# Autodesk Inventor assembly: satu
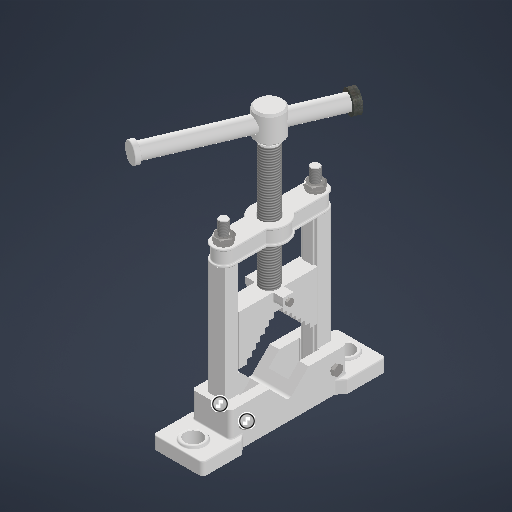
[picture p0: Inventor's stored thumbnail of the model, 512x512]
Saved by Autodesk Inventor 2026.1 (Build 301233000, 233)
## iProperties
Created: 2025-09-15
Part Number: satu
Document SubType Name: Assembly
Designer: student
Author: student
## Documents named in this file (13)
- C:\Users\student\Documents\satu\satu.iam
- C:\Users\student\Documents\satu\alaptest.ipt
- C:\Users\student\Documents\satu\menetesorso.ipt
- C:\Users\student\Documents\satu\oszlop.ipt
- C:\Users\student\Documents\satu\osszekotoelem.ipt
- C:\Users\student\Documents\satu\pfa.ipt
- C:\Users\student\Documents\satu\1.ipt
- C:\Users\student\Documents\Inventor\Content Center Files\R2026\en-US\BS 4464\BS 4464 - 10,6.ipt
- C:\Users\student\Documents\Inventor\Content Center Files\R2026\en-US\DIN 439-2\DIN 439 - M10 x 1,5.ipt
- C:\Users\student\Documents\Inventor\Content Center Files\R2026\en-US\AS 1110\AS 1110 - M6 x 50.ipt
- C:\Users\student\Documents\Inventor\Content Center Files\R2026\en-US\AS 1110\AS 1110 - M4 x 8.ipt
- C:\Users\student\Documents\Inventor\Content Center Files\R2026\en-US\ISO 4034(2)\ISO 4034 - M6 - ISO.ipt
- C:\Users\student\Documents\Inventor\Content Center Files\R2026\en-US\DIN 7989-2\DIN 7989 - 12_ - A.ipt
## Components (18 placed, 12 different names)
1. alaptest:1 — Mate:1, Mate:2, Mate:3, Mate:4, Mate:5, Mate:6, Insert:1, Insert:2, Mate:24, Mate:26
2. menetesorso:1 — Mate:10, Mate:11, Mate:12, Tangent:1, Mate:14
3. oszlop:1 — Mate:1, Mate:2, Mate:3, Mate:7, Mate:9, Mate:15, Mate:21
4. osszekotoelem:1 — Mate:7, Mate:8, Mate:9, Mate:10, Mate:14, Mate:16, Mate:18
5. pfa:1 — Mate:12, Mate:13, Tangent:1, Insert:3, Insert:4
6. 1:1 — Mate:11, Mate:27, Mate:28
7. oszlop:2 — Mate:4, Mate:5, Mate:6, Mate:8, Mate:13, Mate:17, Mate:19
8. BS 4464 10,6:1 — Mate:15, Mate:16, Mate:22
9. BS 4464 10,6:2 — Mate:17, Mate:18, Mate:20
10. DIN 439-2 - replaced by DIN EN 24035/28675 M10:1 — Mate:19, Mate:20
11. DIN 439-2 - replaced by DIN EN 24035/28675 M10:2 — Mate:21, Mate:22
12. AS 1110 - Metric M6 x 50:1 — Insert:1, Mate:25
13. AS 1110 - Metric M6 x 50:2 — Insert:2, Mate:23
14. AS 1110 - Metric M4 x 8:1 — Insert:3
15. AS 1110 - Metric M4 x 8:2 — Insert:4
16. ISO 4034 M6:1 — Mate:23, Mate:24
17. ISO 4034 M6:2 — Mate:25, Mate:26
18. DIN 7989-2 12" - A:1 — Mate:27, Mate:28
## Relationships (33: Mate 28, Insert 4, Tangent 1)
- Mate:1: alaptest:1 ↔ oszlop:1
- Mate:2: alaptest:1 ↔ oszlop:1
- Mate:3: alaptest:1 ↔ oszlop:1
- Mate:4: alaptest:1 ↔ oszlop:2
- Mate:5: alaptest:1 ↔ oszlop:2
- Mate:6: alaptest:1 ↔ oszlop:2
- Mate:7: oszlop:1 ↔ osszekotoelem:1
- Mate:8: osszekotoelem:1 ↔ oszlop:2
- Mate:9: oszlop:1 ↔ osszekotoelem:1
- Mate:10: menetesorso:1 ↔ osszekotoelem:1
- Mate:11: menetesorso:1 ↔ 1:1
- Mate:12: menetesorso:1 ↔ pfa:1
- Mate:13: pfa:1 ↔ oszlop:2
- Tangent:1: menetesorso:1 ↔ pfa:1
- Mate:14 (100 mm): menetesorso:1 ↔ osszekotoelem:1
- Mate:15: oszlop:1 ↔ BS 4464 10,6:1
- Mate:16: osszekotoelem:1 ↔ BS 4464 10,6:1
- Mate:17: oszlop:2 ↔ BS 4464 10,6:2
- Mate:18: osszekotoelem:1 ↔ BS 4464 10,6:2
- Mate:19: oszlop:2 ↔ DIN 439-2 - replaced by DIN EN 24035/28675 M10:1
- Mate:20: BS 4464 10,6:2 ↔ DIN 439-2 - replaced by DIN EN 24035/28675 M10:1
- Mate:21: oszlop:1 ↔ DIN 439-2 - replaced by DIN EN 24035/28675 M10:2
- Mate:22: BS 4464 10,6:1 ↔ DIN 439-2 - replaced by DIN EN 24035/28675 M10:2
- Insert:1: alaptest:1 ↔ AS 1110 - Metric M6 x 50:1
- Insert:2: alaptest:1 ↔ AS 1110 - Metric M6 x 50:2
- Insert:3: pfa:1 ↔ AS 1110 - Metric M4 x 8:1
- Insert:4: pfa:1 ↔ AS 1110 - Metric M4 x 8:2
- Mate:23: AS 1110 - Metric M6 x 50:2 ↔ ISO 4034 M6:1
- Mate:24: alaptest:1 ↔ ISO 4034 M6:1
- Mate:25: AS 1110 - Metric M6 x 50:1 ↔ ISO 4034 M6:2
- Mate:26: alaptest:1 ↔ ISO 4034 M6:2
- Mate:27: 1:1 ↔ DIN 7989-2 12" - A:1
- Mate:28: 1:1 ↔ DIN 7989-2 12" - A:1
